# Autodesk Inventor assembly: Avionics
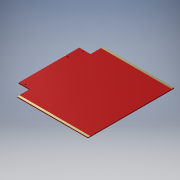
[picture p0: Inventor's stored thumbnail of the model, 180x180]
Saved by Autodesk Inventor 2018 (Build 220112000, 112)
## iProperties
Created: 2018-07-04
Part Number: Avionics
Document SubType Name: Assembly
Designer: Bradley
Author: Bradley
## Documents named in this file (3)
- D:\Users\Bradley\Documents\CougsInSpace\CougSat1-Hardware\CougSat1-AvionicBoard\CADModel\Native\Avionics.iam
- D:\Users\Bradley\Documents\CougsInSpace\CougSat1-Hardware\CougSat1-AvionicBoard\CADModel\Native\Avionics_PCB.ipt
- D:\Users\Bradley\Documents\CougsInSpace\Resources\ComponentModels\Connectors\U.FL_Male.ipt
## Components (2 placed, 2 different names)
1. Avionics_PCB:1 — Mate:1
2. U.FL_Male:1 — Mate:1, Mate:2, Mate:3
## Relationships (3: Mate 3)
- Mate:1: Avionics_PCB:1 ↔ U.FL_Male:1
- Mate:2 (85 mm): U.FL_Male:1
- Mate:3 (15 mm): U.FL_Male:1
